# Autodesk Inventor assembly: smolLipo
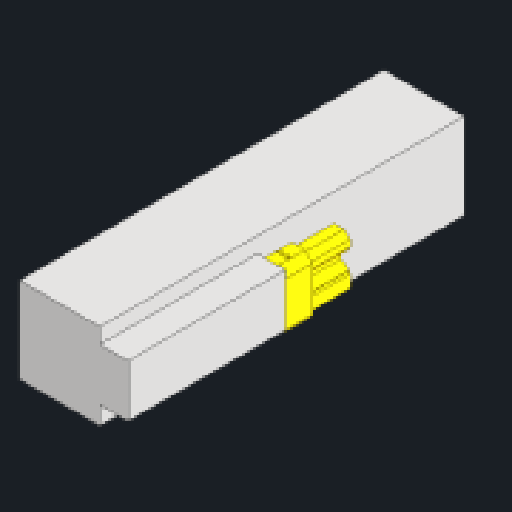
[picture p0: Inventor's stored thumbnail of the model, 512x512]
Saved by Autodesk Inventor 2023 (Build 270158000, 158)
## iProperties
Created: 2024-04-13
Part Number: smolLipo
Document SubType Name: Assembly
Designer: szymo
Mass: 35 g
Surface Area: 58.808 cm^2
Volume: 18.1318 cm^3
Author: szymo
## Documents named in this file (3)
- C:\zRozne\roboilo\robots\wafel\3d_parts\smolLipo.iam
- C:\zRozne\roboilo\robots\wafel\3d_parts\smolLipo.ipt
- C:\zRozne\roboilo\robots\wafel\3d_parts\xt30.ipt
## Components (2 placed, 2 different names)
1. smolLipo:1 — Mate:1, Flush:1, Flush:2
2. xt30:1 — Mate:1, Flush:1, Flush:2
## Relationships (3: Flush 2, Mate 1)
- Mate:1: smolLipo:1 ↔ xt30:1
- Flush:1 (26 mm): smolLipo:1 ↔ xt30:1
- Flush:2 (-2.875 mm): smolLipo:1 ↔ xt30:1
